# Autodesk Inventor assembly: X_rail_Assembly_Rev2
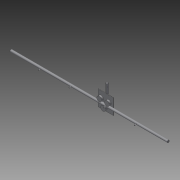
[picture p0: Inventor's stored thumbnail of the model, 180x180]
Saved by Autodesk Inventor 2015 (Build 190159000, 159)
## iProperties
Created: 2016-12-23
Part Number: X_rail_Assembly_Rev2
Document SubType Name: Assembly
Designer: Guy
Mass: 2007.29 g
Surface Area: 3412.18 cm^2
Volume: 2007.29 cm^3
Density: 1 g/cm^3
Author: Guy
## Documents named in this file (4)
- C:\Users\Ernest\Documents\Capstone-Project\doc\CAD\LowLevel_Rev2\X_rail_Assembly_Rev2.iam
- C:\Users\Ernest\Documents\Capstone-Project\doc\CAD\LowLevel_Rev1\X_Rail-Rod-Rev1.ipt
- C:\Users\Ernest\Documents\Capstone-Project\doc\CAD\LowLevel_Rev1\XY_Wheel-Rod-Rev1.ipt
- C:\Users\Ernest\Documents\Capstone-Project\doc\CAD\LowLevel_Rev2\Arm_Base-Rod-Rev2.ipt
## Components (5 placed, 3 different names)
1. X_Rail-Rod-Rev1:1 — Mate:1, Mate:2, Mate:3, Mate:4, Mate:5, Mate:6
2. XY_Wheel-Rod-Rev1:1 — Mate:1, Mate:4, Mate:9
3. XY_Wheel-Rod-Rev1:2 — Mate:2, Mate:5, Mate:7, Mate:8
4. XY_Wheel-Rod-Rev1:3 — Mate:3, Mate:6, Mate:10
5. Arm_Base-Rod-Rev2:1 — Mate:7, Mate:8, Mate:9, Mate:10
## Relationships (10: Mate 10)
- Mate:1: X_Rail-Rod-Rev1:1 ↔ XY_Wheel-Rod-Rev1:1
- Mate:2: X_Rail-Rod-Rev1:1 ↔ XY_Wheel-Rod-Rev1:2
- Mate:3: X_Rail-Rod-Rev1:1 ↔ XY_Wheel-Rod-Rev1:3
- Mate:4 (40 mm): X_Rail-Rod-Rev1:1 ↔ XY_Wheel-Rod-Rev1:1
- Mate:5 (40 mm): X_Rail-Rod-Rev1:1 ↔ XY_Wheel-Rod-Rev1:2
- Mate:6 (-40 mm): X_Rail-Rod-Rev1:1 ↔ XY_Wheel-Rod-Rev1:3
- Mate:7: XY_Wheel-Rod-Rev1:2 ↔ Arm_Base-Rod-Rev2:1
- Mate:8: XY_Wheel-Rod-Rev1:2 ↔ Arm_Base-Rod-Rev2:1
- Mate:9: XY_Wheel-Rod-Rev1:1 ↔ Arm_Base-Rod-Rev2:1
- Mate:10: XY_Wheel-Rod-Rev1:3 ↔ Arm_Base-Rod-Rev2:1
